# Autodesk Inventor assembly: MapleMiniCase_Assembly
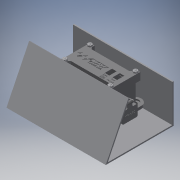
[picture p0: Inventor's stored thumbnail of the model, 180x180]
Saved by Autodesk Inventor 2018 (Build 220112000, 112)
## iProperties
Created: 2019-01-13
Part Number: MapleMiniCase_Assembly
Document SubType Name: Assembly
Designer: tbrow
Author: tbrow
## Documents named in this file (8)
- C:\Users\tbrow\OneDrive\Documents\Arduino1.8.5\MapleMiniCaseCAD\MapleMiniCase_Assembly.iam
- C:\Users\tbrow\OneDrive\Documents\Arduino1.8.5\MapleMiniCaseCAD\KartBuildArea.ipt
- C:\Users\tbrow\OneDrive\Documents\Arduino1.8.5\MapleMiniCaseCAD\MapleMiniCase_Main.ipt
- C:\Users\tbrow\OneDrive\Documents\Arduino\Arduino Case CAD\Reference Models\92220A145_LOW-PROFILE ALLOY STEEL SOCKET HEAD CAP SCREW.ipt
- C:\Users\tbrow\OneDrive\Documents\Arduino\Arduino Case CAD\Reference Models\90633A007_LOW-STRENGTH STEEL THIN NYLON-INSERT LOCKNUT.ipt
- C:\Users\tbrow\OneDrive\Documents\Arduino1.8.5\MapleMiniCaseCAD\SDCardCover.ipt
- C:\Users\tbrow\OneDrive\Documents\Arduino1.8.5\MapleMiniCaseCAD\MMandBatteryCover.ipt
- C:\Users\tbrow\OneDrive\Documents\Arduino1.8.5\MapleMiniCaseCAD\MapleMiniCase_TopCover.ipt
## Components (17 placed, 7 different names)
1. KartBuildArea:1 — Mate:1, Mate:2
2. MapleMiniCase_Main:1 — Mate:1, Insert:1, Insert:2, Insert:3, Insert:4, Insert:5, Insert:6, Insert:7, Angle:1, Insert:8, Insert:9, Insert:10, Insert:11, Mate:2
3. 92220A145_LOW-PROFILE ALLOY STEEL SOCKET HEAD CAP SCREW:1 — Insert:1
4. 92220A145_LOW-PROFILE ALLOY STEEL SOCKET HEAD CAP SCREW:2 — Insert:5
5. 90633A007_LOW-STRENGTH STEEL THIN NYLON-INSERT LOCKNUT:1 — Insert:6
6. 90633A007_LOW-STRENGTH STEEL THIN NYLON-INSERT LOCKNUT:2 — Insert:2
7. SDCardCover:1 — Insert:3
8. MMandBatteryCover:1 — Insert:4
9. MapleMiniCase_TopCover:1 — Insert:7, Angle:1, Insert:12, Insert:13, Insert:14, Insert:15
10. 92220A145_LOW-PROFILE ALLOY STEEL SOCKET HEAD CAP SCREW:3 — Insert:8
11. 92220A145_LOW-PROFILE ALLOY STEEL SOCKET HEAD CAP SCREW:4 — Insert:9
12. 92220A145_LOW-PROFILE ALLOY STEEL SOCKET HEAD CAP SCREW:5 — Insert:10
13. 92220A145_LOW-PROFILE ALLOY STEEL SOCKET HEAD CAP SCREW:6 — Insert:11
14. 90633A007_LOW-STRENGTH STEEL THIN NYLON-INSERT LOCKNUT:3 — Insert:15
15. 90633A007_LOW-STRENGTH STEEL THIN NYLON-INSERT LOCKNUT:4 — Insert:14
16. 90633A007_LOW-STRENGTH STEEL THIN NYLON-INSERT LOCKNUT:5 — Insert:13
17. 90633A007_LOW-STRENGTH STEEL THIN NYLON-INSERT LOCKNUT:6 — Insert:12
## Relationships (18: Insert 15, Mate 2, Angle 1)
- Mate:1 (-69.85 mm): KartBuildArea:1 ↔ MapleMiniCase_Main:1
- Insert:1: MapleMiniCase_Main:1 ↔ 92220A145_LOW-PROFILE ALLOY STEEL SOCKET HEAD CAP SCREW:1
- Insert:2: MapleMiniCase_Main:1 ↔ 90633A007_LOW-STRENGTH STEEL THIN NYLON-INSERT LOCKNUT:2
- Insert:3 (0.508 mm): MapleMiniCase_Main:1 ↔ SDCardCover:1
- Insert:4 (0.508 mm): MapleMiniCase_Main:1 ↔ MMandBatteryCover:1
- Insert:5: MapleMiniCase_Main:1 ↔ 92220A145_LOW-PROFILE ALLOY STEEL SOCKET HEAD CAP SCREW:2
- Insert:6: MapleMiniCase_Main:1 ↔ 90633A007_LOW-STRENGTH STEEL THIN NYLON-INSERT LOCKNUT:1
- Insert:7: MapleMiniCase_Main:1 ↔ MapleMiniCase_TopCover:1
- Angle:1 (0 deg): MapleMiniCase_Main:1 ↔ MapleMiniCase_TopCover:1
- Insert:8: MapleMiniCase_Main:1 ↔ 92220A145_LOW-PROFILE ALLOY STEEL SOCKET HEAD CAP SCREW:3
- Insert:9: MapleMiniCase_Main:1 ↔ 92220A145_LOW-PROFILE ALLOY STEEL SOCKET HEAD CAP SCREW:4
- Insert:10: MapleMiniCase_Main:1 ↔ 92220A145_LOW-PROFILE ALLOY STEEL SOCKET HEAD CAP SCREW:5
- Insert:11: MapleMiniCase_Main:1 ↔ 92220A145_LOW-PROFILE ALLOY STEEL SOCKET HEAD CAP SCREW:6
- Insert:12: MapleMiniCase_TopCover:1 ↔ 90633A007_LOW-STRENGTH STEEL THIN NYLON-INSERT LOCKNUT:6
- Insert:13: MapleMiniCase_TopCover:1 ↔ 90633A007_LOW-STRENGTH STEEL THIN NYLON-INSERT LOCKNUT:5
- Insert:14: MapleMiniCase_TopCover:1 ↔ 90633A007_LOW-STRENGTH STEEL THIN NYLON-INSERT LOCKNUT:4
- Insert:15: MapleMiniCase_TopCover:1 ↔ 90633A007_LOW-STRENGTH STEEL THIN NYLON-INSERT LOCKNUT:3
- Mate:2 (12.7 mm): KartBuildArea:1 ↔ MapleMiniCase_Main:1
